# Autodesk Inventor assembly: Full
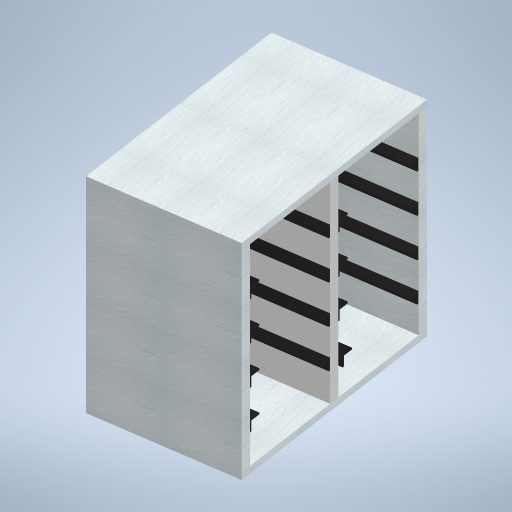
[picture p0: Inventor's stored thumbnail of the model, 512x512]
Saved by Autodesk Inventor 2024.2 (Build 282272000, 272)
## iProperties
Created: 2024-03-09
Part Number: Full
Document SubType Name: Assembly
Designer: lukyv
Author: lukyv
## Documents named in this file (5)
- C:\Users\lukyv\Desktop\Inteligentní inventární systém\3D\Full.iam
- C:\Users\lukyv\Desktop\Inteligentní inventární systém\3D\Deska_bocni.ipt
- C:\Users\lukyv\Desktop\Inteligentní inventární systém\3D\Deska_spodni.ipt
- C:\Users\lukyv\Desktop\Inteligentní inventární systém\3D\BackboardV3.ipt
- C:\Users\lukyv\Desktop\Inteligentní inventární systém\3D\Úhelník.ipt
## Components (31 placed, 4 different names)
1. Deska_bocni:2 — Proti sobě:10, Stejný směr:2, Proti sobě:19, Proti sobě:40, Proti sobě:41, Proti sobě:43, Proti sobě:49, Proti sobě:50, Proti sobě:51, Proti sobě:55, Stejný směr:19
2. Deska_bocni:3 — Proti sobě:11, Proti sobě:12, Proti sobě:15, Proti sobě:16, Proti sobě:20, Proti sobě:21, Proti sobě:22, Proti sobě:23, Proti sobě:26, Proti sobě:29, Proti sobě:39, Proti sobě:44, Proti sobě:45, Proti sobě:46, Proti sobě:47, Stejný směr:16, Stejný směr:17, Proti sobě:48, Proti sobě:54
3. Deska_spodni:2 — Proti sobě:6, Proti sobě:7, Proti sobě:8
4. Deska_bocni:4 — Proti sobě:6, Proti sobě:7, Proti sobě:8, Proti sobě:9, Proti sobě:12, Proti sobě:13, Stejný směr:1, Proti sobě:30, Proti sobě:31, Proti sobě:32, Proti sobě:33, Proti sobě:34, Proti sobě:35, Proti sobě:36, Proti sobě:37
5. Deska_spodni:3 — Proti sobě:9, Proti sobě:10, Proti sobě:11, Proti sobě:17, Stejný směr:1, Stejný směr:2, Proti sobě:18, Proti sobě:19, Stejný směr:15
6. Úhelník:1 — Proti sobě:15, Proti sobě:16, Proti sobě:17, Stejný směr:3, Stejný směr:8
7. Úhelník:2 — Proti sobě:20, Proti sobě:21, Stejný směr:3, Proti sobě:24, Stejný směr:7
8. Úhelník:3 — Proti sobě:22, Proti sobě:23, Proti sobě:24, Stejný směr:4, Stejný směr:6
9. Úhelník:4 — Proti sobě:26, Stejný směr:4, Stejný směr:5, Proti sobě:54
10. Úhelník:5 — Stejný směr:5, Proti sobě:30, Proti sobě:31
11. Úhelník:6 — Stejný směr:6, Proti sobě:32, Proti sobě:33
12. Úhelník:7 — Stejný směr:7, Proti sobě:34, Proti sobě:35
13. Úhelník:8 — Stejný směr:8, Proti sobě:36, Proti sobě:37
14. Úhelník:9 — Proti sobě:43, Proti sobě:49
15. Úhelník:11 — Proti sobě:41, Proti sobě:50, Stejný směr:18
16. Úhelník:12 — Proti sobě:40, Proti sobě:51
17. Úhelník:13 — Proti sobě:39, Proti sobě:47, Proti sobě:48
18. Úhelník:14 — Proti sobě:46, Stejný směr:17
19. Úhelník:15 — Proti sobě:45, Stejný směr:16
20. Úhelník:16 — Proti sobě:44, Stejný směr:15
21. Úhelník:17 — Proti sobě:55, Stejný směr:18, Stejný směr:19
22. BackboardV3:1 — Proti sobě:13, Proti sobě:29
23. BackboardV3:2
24. BackboardV3:3
25. BackboardV3:4
26. BackboardV3:5
27. BackboardV3:6
28. BackboardV3:7
29. BackboardV3:8
30. BackboardV3:9
31. BackboardV3:10
## Component patterns: (10 elements, first: BackboardV3:1)
## Relationships (59: Mate 42, Flush 17)
- Proti sobě:6 [Mate]: Deska_spodni:2 ↔ Deska_bocni:4
- Proti sobě:7 [Mate]: Deska_spodni:2 ↔ Deska_bocni:4
- Proti sobě:8 [Mate]: Deska_spodni:2 ↔ Deska_bocni:4
- Proti sobě:9 [Mate]: Deska_bocni:4 ↔ Deska_spodni:3
- Proti sobě:10 [Mate]: Deska_bocni:2 ↔ Deska_spodni:3
- Proti sobě:11 [Mate]: Deska_bocni:3 ↔ Deska_spodni:3
- Proti sobě:12 [Mate] (173 mm): Deska_bocni:3 ↔ Deska_bocni:4
- Proti sobě:13 [Mate]: Deska_bocni:4 ↔ BackboardV3:1
- Proti sobě:15 [Mate]: Deska_bocni:3 ↔ Úhelník:1
- Proti sobě:16 [Mate]: Deska_bocni:3 ↔ Úhelník:1
- Proti sobě:17 [Mate] (70 mm): Deska_spodni:3 ↔ Úhelník:1
- Stejný směr:1 [Flush]: Deska_bocni:4 ↔ Deska_spodni:3
- Stejný směr:2 [Flush]: Deska_bocni:2 ↔ Deska_spodni:3
- Proti sobě:18 [Mate]: Deska_spodni:3
- Proti sobě:19 [Mate]: Deska_bocni:2 ↔ Deska_spodni:3
- Proti sobě:20 [Mate]: Deska_bocni:3 ↔ Úhelník:2
- Proti sobě:21 [Mate]: Deska_bocni:3 ↔ Úhelník:2
- Stejný směr:3 [Flush] (70 mm): Úhelník:1 ↔ Úhelník:2
- Proti sobě:22 [Mate]: Deska_bocni:3 ↔ Úhelník:3
- Proti sobě:23 [Mate]: Deska_bocni:3 ↔ Úhelník:3
- Proti sobě:24 [Mate] (70 mm): Úhelník:2 ↔ Úhelník:3
- Proti sobě:26 [Mate]: Deska_bocni:3 ↔ Úhelník:4
- Proti sobě:29 [Mate] (14.5 mm): Deska_bocni:3 ↔ BackboardV3:1
- Stejný směr:4 [Flush] (70 mm): Úhelník:3 ↔ Úhelník:4
- Stejný směr:5 [Flush]: Úhelník:4 ↔ Úhelník:5
- Proti sobě:30 [Mate]: Deska_bocni:4 ↔ Úhelník:5
- Proti sobě:31 [Mate]: Deska_bocni:4 ↔ Úhelník:5
- Stejný směr:6 [Flush]: Úhelník:3 ↔ Úhelník:6
- Proti sobě:32 [Mate]: Deska_bocni:4 ↔ Úhelník:6
- Proti sobě:33 [Mate]: Deska_bocni:4 ↔ Úhelník:6
- Stejný směr:7 [Flush]: Úhelník:2 ↔ Úhelník:7
- Proti sobě:34 [Mate]: Deska_bocni:4 ↔ Úhelník:7
- Proti sobě:35 [Mate]: Deska_bocni:4 ↔ Úhelník:7
- Stejný směr:8 [Flush]: Úhelník:1 ↔ Úhelník:8
- Proti sobě:36 [Mate]: Deska_bocni:4 ↔ Úhelník:8
- Proti sobě:37 [Mate]: Deska_bocni:4 ↔ Úhelník:8
- [Flush] (70 mm): Úhelník:11 ↔ Úhelník:12
- [Flush]: Úhelník:12 ↔ Úhelník:13
- [Flush]: Úhelník:11 ↔ Úhelník:14
- [Flush]: Úhelník:9 ↔ Úhelník:16
- Proti sobě:39 [Mate]: Deska_bocni:3 ↔ Úhelník:13
- Proti sobě:40 [Mate]: Deska_bocni:2 ↔ Úhelník:12
- Proti sobě:41 [Mate]: Deska_bocni:2 ↔ Úhelník:11
- Proti sobě:43 [Mate]: Deska_bocni:2 ↔ Úhelník:9
- Proti sobě:44 [Mate]: Deska_bocni:3 ↔ Úhelník:16
- Proti sobě:45 [Mate]: Deska_bocni:3 ↔ Úhelník:15
- Proti sobě:46 [Mate]: Deska_bocni:3 ↔ Úhelník:14
- Proti sobě:47 [Mate]: Deska_bocni:3 ↔ Úhelník:13
- Stejný směr:15 [Flush] (-70 mm): Deska_spodni:3 ↔ Úhelník:16
- Stejný směr:16 [Flush]: Deska_bocni:3 ↔ Úhelník:15
- Stejný směr:17 [Flush]: Deska_bocni:3 ↔ Úhelník:14
- Proti sobě:48 [Mate]: Deska_bocni:3 ↔ Úhelník:13
- Proti sobě:49 [Mate]: Deska_bocni:2 ↔ Úhelník:9
- Proti sobě:50 [Mate]: Deska_bocni:2 ↔ Úhelník:11
- Proti sobě:51 [Mate]: Deska_bocni:2 ↔ Úhelník:12
- Proti sobě:54 [Mate]: Deska_bocni:3 ↔ Úhelník:4
- Proti sobě:55 [Mate]: Deska_bocni:2 ↔ Úhelník:17
- Stejný směr:18 [Flush] (70 mm): Úhelník:11 ↔ Úhelník:17
- Stejný směr:19 [Flush]: Deska_bocni:2 ↔ Úhelník:17
## Named parameters: d60_d54 = 0 mm, d61_d44 = 70 mm, d62_d45 = 0 mm, d63_d48 = 0 mm
